# Autodesk Inventor assembly: Rear Chassis Assembly
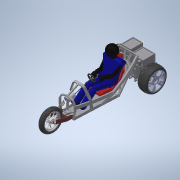
[picture p0: Inventor's stored thumbnail of the model, 180x180]
Saved by Autodesk Inventor 2021 (Build 250183000, 183)
## iProperties
Created: 2020-10-15
Part Number: Rear Chassis Assembly
Document SubType Name: Assembly
Designer: nabee
Author: nabee
## Documents named in this file (22)
- D:\Uni y2\Sem2\236\Design Project\Assembly 4\assembly 4-20201020T195157Z-001\assembly 4\Rear Chassis Assembly.iam
- D:\Uni y2\Sem2\236\Design Project\Assembly 4\assembly 4-20201020T195157Z-001\assembly 4\Motor housing 2.ipt
- D:\Uni y2\Sem2\236\Design Project\Assembly 4\assembly 4-20201020T195157Z-001\assembly 4\Urban Transport Design Project_Master.iam
- D:\Uni y2\Sem2\236\Design Project\Assembly 4\assembly 4-20201020T195157Z-001\assembly 4\Gearbox Housing.ipt
- D:\Uni y2\Sem2\236\Design Project\Assembly 4\assembly 4-20201020T195157Z-001\assembly 4\Differential.ipt
- D:\Uni y2\Sem2\236\Design Project\Assembly 4\assembly 4-20201020T195157Z-001\assembly 4\Diff housing.ipt
- D:\Uni y2\Sem2\236\Design Project\Assembly 4\assembly 4-20201020T195157Z-001\assembly 4\fuel tank housing.ipt
- D:\Uni y2\Sem2\236\Design Project\Assembly 4\assembly 4-20201020T195157Z-001\assembly 4\Engine ktm 690.ipt
- D:\Uni y2\Sem2\236\Design Project\Assembly 4\assembly 4-20201020T195157Z-001\assembly 4\shock absorber.ipt
- D:\Uni y2\Sem2\236\Design Project\Assembly 4\assembly 4-20201020T195157Z-001\assembly 4\Exhaust.ipt
- D:\Uni y2\Sem2\236\Design Project\Assembly 4\assembly 4-20201020T195157Z-001\assembly 4\BakeBrakesAssembly.iam
- D:\Uni y2\Sem2\236\Design Project\Assembly 4\assembly 4-20201020T195157Z-001\assembly 4\Accumulator.ipt
- D:\Uni y2\Sem2\236\Design Project\Assembly 4\assembly 4-20201020T195157Z-001\assembly 4\Gearbox.ipt
- D:\Uni y2\Sem2\236\Design Project\Assembly 4\assembly 4-20201020T195157Z-001\assembly 4\Fuel tank newest.ipt
- D:\Uni y2\Sem2\236\Design Project\Assembly 4\assembly 4-20201020T195157Z-001\assembly 4\Hydraulic Assembly.iam
- D:\Uni y2\Sem2\236\Design Project\Assembly 4\assembly 4-20201020T195157Z-001\assembly 4\Pump and motor Coupled.iam
- D:\Uni y2\Sem2\236\Design Project\Assembly 4\assembly 4-20201020T195157Z-001\assembly 4\support.ipt
- D:\Uni y2\Sem2\236\Design Project\Assembly 4\assembly 4-20201020T195157Z-001\assembly 4\Hydraulic tank.ipt
- D:\Uni y2\Sem2\236\Design Project\Assembly 4\assembly 4-20201020T195157Z-001\assembly 4\connection.ipt
- D:\Uni y2\Sem2\236\Design Project\Assembly 4\assembly 4-20201020T195157Z-001\assembly 4\Spring connection.ipt
- D:\Uni y2\Sem2\236\Design Project\Assembly 4\assembly 4-20201020T195157Z-001\assembly 4\Battery.ipt
- D:\Uni y2\Sem2\236\Design Project\Assembly 4\assembly 4-20201020T195157Z-001\assembly 4\Pump and motor housing new.ipt
## Components (25 placed, 21 different names)
1. Motor housing 2:1 — Mate:2, Flush:2, Flush:3, Mate:3, Mate:4, Mate:8, Mate:9, Mate:10, Rigid:7
2. Urban Transport Design Project_Master:1 [sub-assembly] — Rigid:1, Rotational:2, Rotational:3, Rigid:6
3. Gearbox Housing:1 — Mate:1, Mate:3, Flush:4, Flush:5, Mate:5, Mate:26, Mate:27, Mate:28
4. Differential:1 — Rigid:1, Rigid:2
5. Diff housing:2 — Rigid:2, Mate:1, Mate:2, Flush:2, Flush:3, Flush:4, Mate:34, Flush:7, Mate:35, Flush:8, Tangent:1, Tangent:2, Flush:9, Mate:42, Flush:13, Mate:45, Flush:14
6. fuel tank housing:3 — Flush:5, Mate:4, Mate:5, Mate:29, Mate:30, Mate:31, Mate:43, Flush:12
7. shock absorber:1 — Rotational:8
8. shock absorber:2 — Rotational:10
9. Exhaust:3 — Rigid:5
10. Engine ktm 690:1 — Mate:8, Mate:9, Mate:10, Rigid:5
11. BakeBrakesAssembly:1 [sub-assembly] — Rotational:2, Rotational:7
12. BakeBrakesAssembly:3 [sub-assembly] — Rotational:3, Rotational:9
13. Gearbox:1 — Mate:26, Mate:27, Mate:28
14. Fuel tank newest:1 — Mate:29, Mate:30, Mate:31
15. Hydraulic Assembly:1 [sub-assembly] — Rigid:6, Rigid:8
16. Accumulator:1 — Rigid:7
17. support:1 — Mate:35, Flush:8
18. support:2 — Mate:34, Flush:7
19. Hydraulic tank:1 — Tangent:1, Tangent:2, Flush:9
20. connection:1 — Rigid:8
21. Spring connection:1 — Rotational:7, Rotational:8
22. Spring connection:2 — Rotational:9, Rotational:10
23. Battery:1 — Mate:42, Mate:43, Flush:12
24. Pump and motor Coupled:5 [sub-assembly] — Mate:46, Flush:15
25. Pump and motor housing new:1 — Flush:13, Mate:45, Flush:14, Mate:46, Flush:15
## Relationships (45: Mate 20, Flush 11, WeldJoint 6, RevoluteJoint 6, Tangent 2)
- Rigid:1 [WeldJoint]: Urban Transport Design Project_Master:1 ↔ Differential:1
- Rigid:2 [WeldJoint]: Differential:1 ↔ Diff housing:2
- Mate:1: Gearbox Housing:1 ↔ Diff housing:2
- Mate:2: Motor housing 2:1 ↔ Diff housing:2
- Flush:2: Motor housing 2:1 ↔ Diff housing:2
- Flush:3: Motor housing 2:1 ↔ Diff housing:2
- Mate:3: Motor housing 2:1 ↔ Gearbox Housing:1
- Flush:4: Gearbox Housing:1 ↔ Diff housing:2
- Flush:5: Gearbox Housing:1 ↔ fuel tank housing:3
- Mate:4: Motor housing 2:1 ↔ fuel tank housing:3
- Mate:5: Gearbox Housing:1 ↔ fuel tank housing:3
- Mate:8: Motor housing 2:1 ↔ Engine ktm 690:1
- Mate:9: Motor housing 2:1 ↔ Engine ktm 690:1
- Mate:10: Motor housing 2:1 ↔ Engine ktm 690:1
- Rotational:2 [RevoluteJoint]: Urban Transport Design Project_Master:1 ↔ BakeBrakesAssembly:1
- Rotational:3 [RevoluteJoint]: Urban Transport Design Project_Master:1 ↔ BakeBrakesAssembly:3
- Rigid:5 [WeldJoint]: Exhaust:3 ↔ Engine ktm 690:1
- Mate:26: Gearbox Housing:1 ↔ Gearbox:1
- Mate:27: Gearbox Housing:1 ↔ Gearbox:1
- Mate:28: Gearbox Housing:1 ↔ Gearbox:1
- Mate:29: fuel tank housing:3 ↔ Fuel tank newest:1
- Mate:30: fuel tank housing:3 ↔ Fuel tank newest:1
- Mate:31: fuel tank housing:3 ↔ Fuel tank newest:1
- Rigid:6 [WeldJoint]: Urban Transport Design Project_Master:1 ↔ Hydraulic Assembly:1
- Rigid:7 [WeldJoint]: Motor housing 2:1 ↔ Accumulator:1
- Mate:34: Diff housing:2 ↔ support:2
- Flush:7: Diff housing:2 ↔ support:2
- Mate:35: Diff housing:2 ↔ support:1
- Flush:8: Diff housing:2 ↔ support:1
- Tangent:1: Diff housing:2 ↔ Hydraulic tank:1
- Tangent:2 (17.5 mm): Diff housing:2 ↔ Hydraulic tank:1
- Flush:9 (18.8515 mm): Diff housing:2 ↔ Hydraulic tank:1
- Rigid:8 [WeldJoint]: Hydraulic Assembly:1 ↔ connection:1
- Rotational:7 [RevoluteJoint]: BakeBrakesAssembly:1 ↔ Spring connection:1
- Rotational:8 [RevoluteJoint]: shock absorber:1 ↔ Spring connection:1
- Rotational:9 [RevoluteJoint]: BakeBrakesAssembly:3 ↔ Spring connection:2
- Rotational:10 [RevoluteJoint]: shock absorber:2 ↔ Spring connection:2
- Mate:42: Diff housing:2 ↔ Battery:1
- Mate:43: fuel tank housing:3 ↔ Battery:1
- Flush:12: fuel tank housing:3 ↔ Battery:1
- Flush:13: Diff housing:2 ↔ Pump and motor housing new:1
- Mate:45: Diff housing:2 ↔ Pump and motor housing new:1
- Flush:14: Diff housing:2 ↔ Pump and motor housing new:1
- Mate:46: Pump and motor Coupled:5 ↔ Pump and motor housing new:1
- Flush:15 (5 mm): Pump and motor Coupled:5 ↔ Pump and motor housing new:1
